# Autodesk Inventor assembly: Turdbot Drivetrain
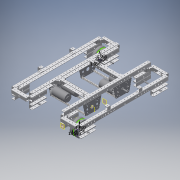
[picture p0: Inventor's stored thumbnail of the model, 180x180]
Saved by Autodesk Inventor 2016 (Build 200138000, 138)
## iProperties
Created: 2016-01-13
Part Number: Turdbot Drivetrain
Document SubType Name: Assembly
Designer: Administrator
Author: Administrator
## Documents named in this file (12)
- C:\Users\Administrator\Desktop\3192CAD\InitialRobotProto\Turdbot Drivetrain.iam
- C:\Users\Administrator\Desktop\3192CAD\InitialRobotProto\DBK_C-Channel_am-2222.ipt
- C:\Users\Administrator\Desktop\3192CAD\InitialRobotProto\DBK_CornerConnect_am-0212.ipt
- C:\Users\Administrator\Desktop\3192CAD\InitialRobotProto\WheelMountStack.iam
- C:\Users\Administrator\Desktop\3192CAD\InitialRobotProto\Wheelaxles.ipt
- C:\Users\Administrator\Desktop\3192CAD\InitialRobotProto\DBK_C-Channel_Tiny.ipt
- C:\Users\Administrator\Desktop\3192CAD\InitialRobotProto\DBK_C-Channel_tenlen.ipt
- C:\Users\Administrator\Desktop\3192CAD\InitialRobotProto\WheelPart.ipt
- C:\Users\Administrator\Desktop\3192CAD\InitialRobotProto\GBPremake\Single.iam
- C:\Users\Administrator\Desktop\3192CAD\InitialRobotProto\GBPremake\Single_d02.ipt
- C:\Users\Administrator\Desktop\3192CAD\InitialRobotProto\DBK_CrossHexTube_am-2241.ipt
- C:\Users\Administrator\Desktop\3192CAD\InitialRobotProto\niblet.ipt
## Components (52 placed, 11 different names)
1. DBK_C-Channel_am-2222:1 — Mate:1, Mate:2, Mate:3, Mate:16, Mate:17, Mate:18, Mate:40, Mate:41, Mate:42, Mate:43, Mate:44, Mate:45, Mate:197, Mate:198, Mate:201, Mate:202, Flush:4, Flush:5
2. DBK_C-Channel_am-2222:4 — Mate:10, Mate:11, Mate:12, Mate:13, Mate:14, Mate:15, Mate:52, Mate:53, Mate:54, Mate:55, Mate:56, Mate:57, Mate:199, Mate:200, Mate:203, Mate:204, Flush:2, Flush:3
3. DBK_CornerConnect_am-0212:1 — Mate:10, Mate:11, Mate:12, Mate:106, Mate:107, Mate:163
4. DBK_CornerConnect_am-0212:2 — Mate:16, Mate:17, Mate:18, Mate:91, Mate:93
5. DBK_CornerConnect_am-0212:3 — Mate:1, Mate:2, Mate:3, Mate:94, Mate:96, Mate:98
6. DBK_CornerConnect_am-0212:4 — Mate:13, Mate:14, Mate:15, Mate:101, Mate:102, Mate:157
7. WheelMountStack:1 [sub-assembly] — Mate:55, Mate:56, Mate:57, Mate:60
8. WheelMountStack:2 [sub-assembly] — Mate:52, Mate:53, Mate:54, Mate:59
9. WheelMountStack:6 [sub-assembly] — Mate:43, Mate:44, Mate:45, Mate:144
10. WheelMountStack:7 [sub-assembly] — Mate:40, Mate:41, Mate:42, Mate:187
11. Wheelaxles:1 — Mate:143, Mate:144
12. Wheelaxles:2 — Mate:59
13. Wheelaxles:3 — Mate:60, Mate:188
14. Wheelaxles:4 — Mate:187
15. DBK_C-Channel_am-2222:5 — Mate:124, Mate:125, Mate:126, Mate:127, Mate:128, Mate:129, Mate:145, Mate:146, Mate:147, Mate:154, Mate:155, Mate:156, Mate:166, Mate:167, Mate:168, Mate:169, Mate:171
16. DBK_C-Channel_Tiny:1 — Mate:73, Mate:74, Mate:75, Mate:164, Mate:165, Mate:178, Mate:179, Mate:180
17. DBK_C-Channel_Tiny:2 — Mate:82, Mate:83, Mate:84, Mate:168, Mate:169, Mate:172, Mate:173, Mate:174
18. DBK_C-Channel_Tiny:3 — Mate:76, Mate:77, Mate:78, Mate:160, Mate:161, Mate:162, Mate:181, Mate:182, Mate:183
19. DBK_C-Channel_Tiny:4 — Mate:79, Mate:80, Mate:81, Mate:166, Mate:167, Mate:171, Mate:184, Mate:185, Mate:186
20. DBK_CornerConnect_am-0212:5 — Mate:76, Mate:77, Mate:78, Mate:99, Mate:100, Mate:103
21. DBK_CornerConnect_am-0212:6 — Mate:82, Mate:83, Mate:84, Mate:95, Mate:97, Mate:159
22. DBK_CornerConnect_am-0212:7 — Mate:73, Mate:74, Mate:75, Mate:104, Mate:105, Mate:108
23. DBK_CornerConnect_am-0212:8 — Mate:79, Mate:80, Mate:81, Mate:92, Mate:158, Mate:170
24. DBK_CornerConnect_am-0212:9 — Mate:121, Mate:122, Mate:123, Mate:138, Mate:139
25. DBK_CornerConnect_am-0212:10 — Mate:124, Mate:125, Mate:126, Mate:140, Mate:141, Mate:142
26. DBK_CornerConnect_am-0212:11 — Mate:130, Mate:131, Mate:132, Mate:135, Mate:136, Mate:137
27. DBK_CornerConnect_am-0212:12 — Mate:127, Mate:128, Mate:129, Mate:133, Mate:134
28. DBK_C-Channel_am-2222:6 — Mate:121, Mate:122, Mate:123, Mate:130, Mate:131, Mate:132, Mate:148, Mate:149, Mate:150, Mate:151, Mate:152, Mate:153, Mate:160, Mate:161, Mate:162, Mate:164, Mate:165
29. DBK_C-Channel_Tiny:5 — Mate:94, Mate:95, Mate:96, Mate:97, Mate:98, Mate:159
30. DBK_C-Channel_Tiny:6 — Mate:104, Mate:105, Mate:106, Mate:107, Mate:108, Mate:163
31. DBK_C-Channel_Tiny:7 — Mate:99, Mate:100, Mate:101, Mate:102, Mate:103, Mate:157
32. DBK_C-Channel_Tiny:8 — Mate:91, Mate:92, Mate:93, Mate:158, Mate:170
33. DBK_C-Channel_tenlen:1 — Mate:133, Mate:134, Mate:135, Mate:136, Mate:137
34. DBK_C-Channel_tenlen:2 — Mate:138, Mate:139, Mate:140, Mate:141, Mate:142
35. WheelPart:1 — Mate:143
36. WheelPart:2 — Mate:188
37. Single:1 [sub-assembly] — Mate:145, Mate:146, Mate:147, Mate:189, Mate:190, Mate:195
38. Single:2 [sub-assembly] — Mate:148, Mate:149, Mate:150
39. Single_d02:1 — Mate:154, Mate:155, Mate:156, Mate:191, Mate:192, Mate:193, Mate:194
40. Single_d02:2 — Mate:151, Mate:152, Mate:153, Mate:196
41. WheelMountStack:8 [sub-assembly] — Mate:172, Mate:173, Mate:174
42. WheelMountStack:10 [sub-assembly] — Mate:181, Mate:182, Mate:183, Flush:1
43. WheelMountStack:11 [sub-assembly] — Mate:178, Mate:179, Mate:180
44. WheelMountStack:12 [sub-assembly] — Mate:184, Mate:185, Mate:186
45. DBK_CrossHexTube_am-2241:1 — Mate:191, Mate:192
46. DBK_CrossHexTube_am-2241:2 — Mate:189, Mate:190, Flush:1
47. DBK_CrossHexTube_am-2241:3 — Mate:195, Mate:196
48. DBK_CrossHexTube_am-2241:4 — Mate:193, Mate:194
49. niblet:1 — Mate:197, Mate:201, Flush:4
50. niblet:2 — Mate:198, Mate:202, Flush:5
51. niblet:3 — Mate:199, Mate:203, Flush:3
52. niblet:4 — Mate:200, Mate:204, Flush:2
## Relationships (142: Mate 137, Flush 5)
- Mate:1: DBK_C-Channel_am-2222:1 ↔ DBK_CornerConnect_am-0212:3
- Mate:2: DBK_C-Channel_am-2222:1 ↔ DBK_CornerConnect_am-0212:3
- Mate:3: DBK_C-Channel_am-2222:1 ↔ DBK_CornerConnect_am-0212:3
- Mate:10: DBK_C-Channel_am-2222:4 ↔ DBK_CornerConnect_am-0212:1
- Mate:11: DBK_C-Channel_am-2222:4 ↔ DBK_CornerConnect_am-0212:1
- Mate:12: DBK_C-Channel_am-2222:4 ↔ DBK_CornerConnect_am-0212:1
- Mate:13: DBK_C-Channel_am-2222:4 ↔ DBK_CornerConnect_am-0212:4
- Mate:14: DBK_C-Channel_am-2222:4 ↔ DBK_CornerConnect_am-0212:4
- Mate:15: DBK_C-Channel_am-2222:4 ↔ DBK_CornerConnect_am-0212:4
- Mate:16: DBK_C-Channel_am-2222:1 ↔ DBK_CornerConnect_am-0212:2
- Mate:17: DBK_C-Channel_am-2222:1 ↔ DBK_CornerConnect_am-0212:2
- Mate:18: DBK_C-Channel_am-2222:1 ↔ DBK_CornerConnect_am-0212:2
- Mate:40: DBK_C-Channel_am-2222:1 ↔ WheelMountStack:7
- Mate:41: DBK_C-Channel_am-2222:1 ↔ WheelMountStack:7
- Mate:42: DBK_C-Channel_am-2222:1 ↔ WheelMountStack:7
- Mate:43: DBK_C-Channel_am-2222:1 ↔ WheelMountStack:6
- Mate:44: DBK_C-Channel_am-2222:1 ↔ WheelMountStack:6
- Mate:45: DBK_C-Channel_am-2222:1 ↔ WheelMountStack:6
- Mate:52: DBK_C-Channel_am-2222:4 ↔ WheelMountStack:2
- Mate:53: DBK_C-Channel_am-2222:4 ↔ WheelMountStack:2
- Mate:54: DBK_C-Channel_am-2222:4 ↔ WheelMountStack:2
- Mate:55: DBK_C-Channel_am-2222:4 ↔ WheelMountStack:1
- Mate:56: DBK_C-Channel_am-2222:4 ↔ WheelMountStack:1
- Mate:57: DBK_C-Channel_am-2222:4 ↔ WheelMountStack:1
- Mate:59: WheelMountStack:2 ↔ Wheelaxles:2
- Mate:60: WheelMountStack:1 ↔ Wheelaxles:3
- Mate:73: DBK_C-Channel_Tiny:1 ↔ DBK_CornerConnect_am-0212:7
- Mate:74: DBK_C-Channel_Tiny:1 ↔ DBK_CornerConnect_am-0212:7
- Mate:75: DBK_C-Channel_Tiny:1 ↔ DBK_CornerConnect_am-0212:7
- Mate:76: DBK_C-Channel_Tiny:3 ↔ DBK_CornerConnect_am-0212:5
- Mate:77: DBK_C-Channel_Tiny:3 ↔ DBK_CornerConnect_am-0212:5
- Mate:78: DBK_C-Channel_Tiny:3 ↔ DBK_CornerConnect_am-0212:5
- Mate:79: DBK_C-Channel_Tiny:4 ↔ DBK_CornerConnect_am-0212:8
- Mate:80: DBK_C-Channel_Tiny:4 ↔ DBK_CornerConnect_am-0212:8
- Mate:81: DBK_C-Channel_Tiny:4 ↔ DBK_CornerConnect_am-0212:8
- Mate:82: DBK_C-Channel_Tiny:2 ↔ DBK_CornerConnect_am-0212:6
- Mate:83: DBK_C-Channel_Tiny:2 ↔ DBK_CornerConnect_am-0212:6
- Mate:84: DBK_C-Channel_Tiny:2 ↔ DBK_CornerConnect_am-0212:6
- Mate:91: DBK_CornerConnect_am-0212:2 ↔ DBK_C-Channel_Tiny:8
- Mate:92: DBK_CornerConnect_am-0212:8 ↔ DBK_C-Channel_Tiny:8
- Mate:93: DBK_CornerConnect_am-0212:2 ↔ DBK_C-Channel_Tiny:8
- Mate:94: DBK_CornerConnect_am-0212:3 ↔ DBK_C-Channel_Tiny:5
- Mate:95: DBK_CornerConnect_am-0212:6 ↔ DBK_C-Channel_Tiny:5
- Mate:96: DBK_CornerConnect_am-0212:3 ↔ DBK_C-Channel_Tiny:5
- Mate:97: DBK_CornerConnect_am-0212:6 ↔ DBK_C-Channel_Tiny:5
- Mate:98: DBK_CornerConnect_am-0212:3 ↔ DBK_C-Channel_Tiny:5
- Mate:99: DBK_CornerConnect_am-0212:5 ↔ DBK_C-Channel_Tiny:7
- Mate:100: DBK_CornerConnect_am-0212:5 ↔ DBK_C-Channel_Tiny:7
- Mate:101: DBK_CornerConnect_am-0212:4 ↔ DBK_C-Channel_Tiny:7
- Mate:102: DBK_CornerConnect_am-0212:4 ↔ DBK_C-Channel_Tiny:7
- Mate:103: DBK_CornerConnect_am-0212:5 ↔ DBK_C-Channel_Tiny:7
- Mate:104: DBK_CornerConnect_am-0212:7 ↔ DBK_C-Channel_Tiny:6
- Mate:105: DBK_CornerConnect_am-0212:7 ↔ DBK_C-Channel_Tiny:6
- Mate:106: DBK_CornerConnect_am-0212:1 ↔ DBK_C-Channel_Tiny:6
- Mate:107: DBK_CornerConnect_am-0212:1 ↔ DBK_C-Channel_Tiny:6
- Mate:108: DBK_CornerConnect_am-0212:7 ↔ DBK_C-Channel_Tiny:6
- Mate:121: DBK_CornerConnect_am-0212:9 ↔ DBK_C-Channel_am-2222:6
- Mate:122: DBK_CornerConnect_am-0212:9 ↔ DBK_C-Channel_am-2222:6
- Mate:123: DBK_CornerConnect_am-0212:9 ↔ DBK_C-Channel_am-2222:6
- Mate:124: DBK_C-Channel_am-2222:5 ↔ DBK_CornerConnect_am-0212:10
- Mate:125: DBK_C-Channel_am-2222:5 ↔ DBK_CornerConnect_am-0212:10
- Mate:126: DBK_C-Channel_am-2222:5 ↔ DBK_CornerConnect_am-0212:10
- Mate:127: DBK_C-Channel_am-2222:5 ↔ DBK_CornerConnect_am-0212:12
- Mate:128: DBK_C-Channel_am-2222:5 ↔ DBK_CornerConnect_am-0212:12
- Mate:129: DBK_C-Channel_am-2222:5 ↔ DBK_CornerConnect_am-0212:12
- Mate:130: DBK_CornerConnect_am-0212:11 ↔ DBK_C-Channel_am-2222:6
- Mate:131: DBK_CornerConnect_am-0212:11 ↔ DBK_C-Channel_am-2222:6
- Mate:132: DBK_CornerConnect_am-0212:11 ↔ DBK_C-Channel_am-2222:6
- Mate:133: DBK_CornerConnect_am-0212:12 ↔ DBK_C-Channel_tenlen:1
- Mate:134: DBK_CornerConnect_am-0212:12 ↔ DBK_C-Channel_tenlen:1
- Mate:135: DBK_CornerConnect_am-0212:11 ↔ DBK_C-Channel_tenlen:1
- Mate:136: DBK_CornerConnect_am-0212:11 ↔ DBK_C-Channel_tenlen:1
- Mate:137: DBK_CornerConnect_am-0212:11 ↔ DBK_C-Channel_tenlen:1
- Mate:138: DBK_CornerConnect_am-0212:9 ↔ DBK_C-Channel_tenlen:2
- Mate:139: DBK_CornerConnect_am-0212:9 ↔ DBK_C-Channel_tenlen:2
- Mate:140: DBK_CornerConnect_am-0212:10 ↔ DBK_C-Channel_tenlen:2
- Mate:141: DBK_CornerConnect_am-0212:10 ↔ DBK_C-Channel_tenlen:2
- Mate:142: DBK_CornerConnect_am-0212:10 ↔ DBK_C-Channel_tenlen:2
- Mate:143: Wheelaxles:1 ↔ WheelPart:1
- Mate:144: WheelMountStack:6 ↔ Wheelaxles:1
- Mate:145: DBK_C-Channel_am-2222:5 ↔ Single:1
- Mate:146: DBK_C-Channel_am-2222:5 ↔ Single:1
- Mate:147: DBK_C-Channel_am-2222:5 ↔ Single:1
- Mate:148: DBK_C-Channel_am-2222:6 ↔ Single:2
- Mate:149: DBK_C-Channel_am-2222:6 ↔ Single:2
- Mate:150: DBK_C-Channel_am-2222:6 ↔ Single:2
- Mate:151: DBK_C-Channel_am-2222:6 ↔ Single_d02:2
- Mate:152: DBK_C-Channel_am-2222:6 ↔ Single_d02:2
- Mate:153: DBK_C-Channel_am-2222:6 ↔ Single_d02:2
- Mate:154: DBK_C-Channel_am-2222:5 ↔ Single_d02:1
- Mate:155: DBK_C-Channel_am-2222:5 ↔ Single_d02:1
- Mate:156: DBK_C-Channel_am-2222:5 ↔ Single_d02:1
- Mate:157: DBK_CornerConnect_am-0212:4 ↔ DBK_C-Channel_Tiny:7
- Mate:158: DBK_CornerConnect_am-0212:8 ↔ DBK_C-Channel_Tiny:8
- Mate:159: DBK_CornerConnect_am-0212:6 ↔ DBK_C-Channel_Tiny:5
- Mate:160: DBK_C-Channel_Tiny:3 ↔ DBK_C-Channel_am-2222:6
- Mate:161: DBK_C-Channel_Tiny:3 ↔ DBK_C-Channel_am-2222:6
- Mate:162: DBK_C-Channel_Tiny:3 ↔ DBK_C-Channel_am-2222:6
- Mate:163: DBK_CornerConnect_am-0212:1 ↔ DBK_C-Channel_Tiny:6
- Mate:164: DBK_C-Channel_Tiny:1 ↔ DBK_C-Channel_am-2222:6
- Mate:165: DBK_C-Channel_Tiny:1 ↔ DBK_C-Channel_am-2222:6
- Mate:166: DBK_C-Channel_am-2222:5 ↔ DBK_C-Channel_Tiny:4
- Mate:167: DBK_C-Channel_am-2222:5 ↔ DBK_C-Channel_Tiny:4
- Mate:168: DBK_C-Channel_am-2222:5 ↔ DBK_C-Channel_Tiny:2
- Mate:169: DBK_C-Channel_am-2222:5 ↔ DBK_C-Channel_Tiny:2
- Mate:170: DBK_CornerConnect_am-0212:8 ↔ DBK_C-Channel_Tiny:8
- Mate:171: DBK_C-Channel_am-2222:5 ↔ DBK_C-Channel_Tiny:4
- Mate:172: DBK_C-Channel_Tiny:2 ↔ WheelMountStack:8
- Mate:173: DBK_C-Channel_Tiny:2 ↔ WheelMountStack:8
- Mate:174: DBK_C-Channel_Tiny:2 ↔ WheelMountStack:8
- Mate:178: DBK_C-Channel_Tiny:1 ↔ WheelMountStack:11
- Mate:179: DBK_C-Channel_Tiny:1 ↔ WheelMountStack:11
- Mate:180: DBK_C-Channel_Tiny:1 ↔ WheelMountStack:11
- Mate:181: DBK_C-Channel_Tiny:3 ↔ WheelMountStack:10
- Mate:182: DBK_C-Channel_Tiny:3 ↔ WheelMountStack:10
- Mate:183: DBK_C-Channel_Tiny:3 ↔ WheelMountStack:10
- Mate:184: DBK_C-Channel_Tiny:4 ↔ WheelMountStack:12
- Mate:185: DBK_C-Channel_Tiny:4 ↔ WheelMountStack:12
- Mate:186: DBK_C-Channel_Tiny:4 ↔ WheelMountStack:12
- Mate:187: WheelMountStack:7 ↔ Wheelaxles:4
- Mate:188: Wheelaxles:3 ↔ WheelPart:2
- Mate:189: Single:1 ↔ DBK_CrossHexTube_am-2241:2
- Mate:190: Single:1 ↔ DBK_CrossHexTube_am-2241:2
- Mate:191: Single_d02:1 ↔ DBK_CrossHexTube_am-2241:1
- Mate:192: Single_d02:1 ↔ DBK_CrossHexTube_am-2241:1
- Flush:1: WheelMountStack:10 ↔ DBK_CrossHexTube_am-2241:2
- Mate:193: Single_d02:1 ↔ DBK_CrossHexTube_am-2241:4
- Mate:194: Single_d02:1 ↔ DBK_CrossHexTube_am-2241:4
- Mate:195: Single:1 ↔ DBK_CrossHexTube_am-2241:3
- Mate:196: Single_d02:2 ↔ DBK_CrossHexTube_am-2241:3
- Mate:197: DBK_C-Channel_am-2222:1 ↔ niblet:1
- Mate:198: DBK_C-Channel_am-2222:1 ↔ niblet:2
- Mate:199: DBK_C-Channel_am-2222:4 ↔ niblet:3
- Mate:200: DBK_C-Channel_am-2222:4 ↔ niblet:4
- Mate:201: DBK_C-Channel_am-2222:1 ↔ niblet:1
- Mate:202: DBK_C-Channel_am-2222:1 ↔ niblet:2
- Mate:203: DBK_C-Channel_am-2222:4 ↔ niblet:3
- Mate:204: DBK_C-Channel_am-2222:4 ↔ niblet:4
- Flush:2: DBK_C-Channel_am-2222:4 ↔ niblet:4
- Flush:3: DBK_C-Channel_am-2222:4 ↔ niblet:3
- Flush:4: DBK_C-Channel_am-2222:1 ↔ niblet:1
- Flush:5: DBK_C-Channel_am-2222:1 ↔ niblet:2
